# Autodesk Inventor assembly: 3DCP-SYSTEM
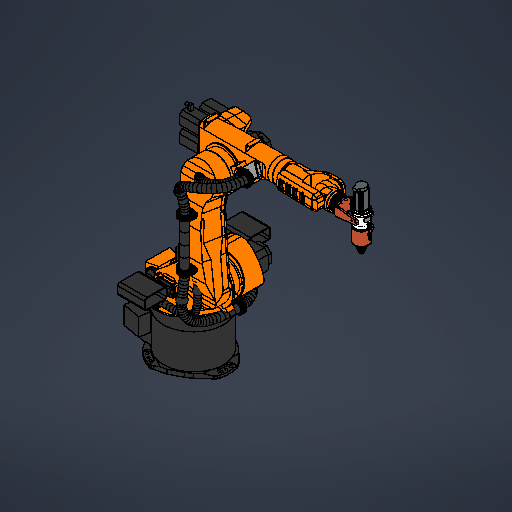
[picture p0: Inventor's stored thumbnail of the model, 512x512]
Saved by Autodesk Inventor 2025.3 (Build 293356030, 356C)
## iProperties
Created: 2025-09-03
Part Number: 3DCP-SYSTEM
Document SubType Name: Assembly
Designer: lstk1ng
Author: lstk1ng
## Documents named in this file (3)
- C:\Users\lstk1ng\Documents\UPC\UPC-10\PROYECTO MECATRONICO 1\3DCP-SYSTEM.iam
- C:\Users\lstk1ng\Documents\UPC\UPC-10\PROYECTO MECATRONICO 1\KUKA KR 60-3\KR60-3.ipt
- C:\Users\lstk1ng\Documents\UPC\UPC-10\PROYECTO MECATRONICO 1\3DCP-NOZZLE.iam
## Components (2 placed, 2 different names)
1. KR60-3:1 — Mate:1, Mate:2
2. 3DCP-NOZZLE:1 [sub-assembly] — Mate:1, Mate:2
## Relationships (2: Mate 2)
- Mate:1: KR60-3:1 ↔ 3DCP-NOZZLE:1
- Mate:2: KR60-3:1 ↔ 3DCP-NOZZLE:1
